# Autodesk Inventor assembly: 000 ASY GBK Gubkinskiy
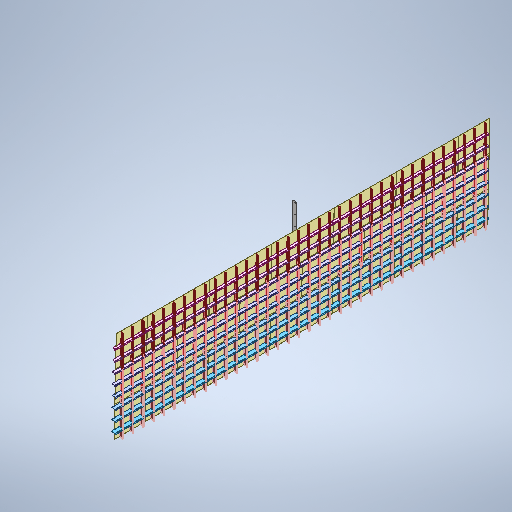
[picture p0: Inventor's stored thumbnail of the model, 512x512]
Saved by Autodesk Inventor 2026.2 (Build 302298000, 298)
## iProperties
Created: 2026-04-17
Part Number: 000 ASY GBK Gubkinskiy
Document SubType Name: Assembly
Designer: admin
Author: admin
## Documents named in this file (13)
- C:\Users\admin\Documents\Inventor\GBK-Gubkinskiy\000 ASY GBK Gubkinskiy.iam
- C:\Users\admin\Documents\Inventor\GBK-Gubkinskiy\GBK bottom.ipt
- C:\Users\admin\Documents\Inventor\GBK-Gubkinskiy\01 ASY GBK wall shield 1.1.1.iam
- C:\Users\admin\Documents\Inventor\GBK-Gubkinskiy\GBK dummy wall 1.ipt
- C:\Users\admin\Documents\Inventor\GBK-Gubkinskiy\GBK dummy wall 4.ipt
- C:\Users\admin\Documents\Inventor\GBK-Gubkinskiy\GBK overall model.ipt
- C:\Users\admin\Documents\Inventor\GBK-Gubkinskiy\02.1 GBK main rib.ipt
- C:\Users\admin\Documents\Inventor\GBK-Gubkinskiy\03.1 GBK main3  rib.ipt
- C:\Users\admin\Documents\Inventor\GBK-Gubkinskiy\02 ASY GBK wall shield 1.1.2.iam
- C:\Users\admin\Documents\Inventor\GBK-Gubkinskiy\04 ASY GBK wall shield 1.2.4.iam
- C:\Users\admin\Documents\Inventor\GBK-Gubkinskiy\07 ASY GBK wall shield 1.3.1.iam
- C:\Users\admin\Documents\Inventor\GBK-Gubkinskiy\08 ASY GBK wall shield 1.3.8.iam
- C:\Users\admin\Documents\Inventor\GBK-Gubkinskiy\0411 GBK Center main rib.ipt
## Components (28 placed, 13 different names)
1. GBK bottom.ipt:1 — Mate:10, Mate:11, Mate:12, Mate:13, Mate:14, Rigid:1
2. 01 ASY GBK wall shield 1.1.1.iam:1 [sub-assembly] — Rigid:4, Rigid:5
3. GBK dummy wall 1.ipt:1 — Mate:10
4. GBK dummy wall 1.ipt:2 — Mate:11, Mate:12
5. GBK dummy wall 4.ipt:1 — Mate:13, Mate:14
6. GBK overall model:1 — Rigid:1
7. 02.1 GBK main rib:1 — Rigid:3
8. 03.1 GBK main3  rib:1 — Rigid:3
9. 02 ASY GBK wall shield 1.1.2:1 [sub-assembly] — Rigid:4, Rigid:17
10. 04 ASY GBK wall shield 1.2.4:1 [sub-assembly] — Rigid:5, Rigid:6, Rigid:12
11. 07 ASY GBK wall shield 1.3.1:1 [sub-assembly] — Rigid:6, Rigid:7
12. 08 ASY GBK wall shield 1.3.8:1 [sub-assembly] — Rigid:7, Rigid:8
13. 08 ASY GBK wall shield 1.3.8:2 [sub-assembly] — Rigid:8, Rigid:9
14. 08 ASY GBK wall shield 1.3.8:3 [sub-assembly] — Rigid:9, Rigid:10
15. 08 ASY GBK wall shield 1.3.8:4 [sub-assembly] — Rigid:10, Rigid:11
16. 08 ASY GBK wall shield 1.3.8:5 [sub-assembly] — Rigid:11, Rigid:22
17. 04 ASY GBK wall shield 1.2.4:2 [sub-assembly] — Rigid:12, Rigid:13
18. 04 ASY GBK wall shield 1.2.4:3 [sub-assembly] — Rigid:13, Rigid:14
19. 04 ASY GBK wall shield 1.2.4:4 [sub-assembly] — Rigid:14, Rigid:15
20. 04 ASY GBK wall shield 1.2.4:5 [sub-assembly] — Rigid:15, Rigid:16
21. 04 ASY GBK wall shield 1.2.4:6 [sub-assembly] — Rigid:16
22. 02 ASY GBK wall shield 1.1.2:2 [sub-assembly] — Rigid:17, Rigid:18
23. 02 ASY GBK wall shield 1.1.2:3 [sub-assembly] — Rigid:18, Rigid:19
24. 02 ASY GBK wall shield 1.1.2:4 [sub-assembly] — Rigid:19, Rigid:20
25. 02 ASY GBK wall shield 1.1.2:5 [sub-assembly] — Rigid:20, Rigid:21
26. 01 ASY GBK wall shield 1.1.1:2 [sub-assembly] — Rigid:21
27. 07 ASY GBK wall shield 1.3.1:2 [sub-assembly] — Rigid:22
28. 0411 GBK Center main rib:1
## Relationships (30: WeldJoint 21, Mate 6, Flush 2, RevoluteJoint 1)
- [Flush]: GBK bottom.ipt:1 ↔ 01 ASY GBK wall shield 1.1.1.iam:1
- [Mate]: GBK bottom.ipt:1 ↔ 01 ASY GBK wall shield 1.1.1.iam:1
- Mate:10: GBK bottom.ipt:1 ↔ GBK dummy wall 1.ipt:1
- Mate:11: GBK bottom.ipt:1 ↔ GBK dummy wall 1.ipt:2
- Mate:12: GBK bottom.ipt:1 ↔ GBK dummy wall 1.ipt:2
- Mate:13: GBK bottom.ipt:1 ↔ GBK dummy wall 4.ipt:1
- Mate:14: GBK bottom.ipt:1 ↔ GBK dummy wall 4.ipt:1
- Rigid:1 [WeldJoint]: GBK bottom.ipt:1 ↔ GBK overall model:1
- [RevoluteJoint]: 01 ASY GBK wall shield 1.1.1.iam:1 ↔ 02.1 GBK main rib:1
- Rigid:3 [WeldJoint]: 02.1 GBK main rib:1 ↔ 03.1 GBK main3  rib:1
- [Flush]: 01 ASY GBK wall shield 1.1.1.iam:1 ↔ 02.1 GBK main rib:1
- Rigid:4 [WeldJoint] (1 mm): 01 ASY GBK wall shield 1.1.1.iam:1 ↔ 02 ASY GBK wall shield 1.1.2:1
- Rigid:5 [WeldJoint]: 01 ASY GBK wall shield 1.1.1.iam:1 ↔ 04 ASY GBK wall shield 1.2.4:1
- Rigid:6 [WeldJoint]: 04 ASY GBK wall shield 1.2.4:1 ↔ 07 ASY GBK wall shield 1.3.1:1
- Rigid:7 [WeldJoint] (1 mm): 07 ASY GBK wall shield 1.3.1:1 ↔ 08 ASY GBK wall shield 1.3.8:1
- Rigid:8 [WeldJoint] (1 mm): 08 ASY GBK wall shield 1.3.8:1 ↔ 08 ASY GBK wall shield 1.3.8:2
- Rigid:9 [WeldJoint] (1 mm): 08 ASY GBK wall shield 1.3.8:2 ↔ 08 ASY GBK wall shield 1.3.8:3
- Rigid:10 [WeldJoint] (1 mm): 08 ASY GBK wall shield 1.3.8:3 ↔ 08 ASY GBK wall shield 1.3.8:4
- Rigid:11 [WeldJoint] (1 mm): 08 ASY GBK wall shield 1.3.8:4 ↔ 08 ASY GBK wall shield 1.3.8:5
- Rigid:12 [WeldJoint] (1 mm): 04 ASY GBK wall shield 1.2.4:1 ↔ 04 ASY GBK wall shield 1.2.4:2
- Rigid:13 [WeldJoint] (1 mm): 04 ASY GBK wall shield 1.2.4:2 ↔ 04 ASY GBK wall shield 1.2.4:3
- Rigid:14 [WeldJoint] (1 mm): 04 ASY GBK wall shield 1.2.4:3 ↔ 04 ASY GBK wall shield 1.2.4:4
- Rigid:15 [WeldJoint] (1 mm): 04 ASY GBK wall shield 1.2.4:4 ↔ 04 ASY GBK wall shield 1.2.4:5
- Rigid:16 [WeldJoint] (1 mm): 04 ASY GBK wall shield 1.2.4:5 ↔ 04 ASY GBK wall shield 1.2.4:6
- Rigid:17 [WeldJoint] (1 mm): 02 ASY GBK wall shield 1.1.2:1 ↔ 02 ASY GBK wall shield 1.1.2:2
- Rigid:18 [WeldJoint] (1 mm): 02 ASY GBK wall shield 1.1.2:2 ↔ 02 ASY GBK wall shield 1.1.2:3
- Rigid:19 [WeldJoint] (1 mm): 02 ASY GBK wall shield 1.1.2:3 ↔ 02 ASY GBK wall shield 1.1.2:4
- Rigid:20 [WeldJoint] (1 mm): 02 ASY GBK wall shield 1.1.2:4 ↔ 02 ASY GBK wall shield 1.1.2:5
- Rigid:21 [WeldJoint] (1 mm): 02 ASY GBK wall shield 1.1.2:5 ↔ 01 ASY GBK wall shield 1.1.1:2
- Rigid:22 [WeldJoint] (1 mm): 08 ASY GBK wall shield 1.3.8:5 ↔ 07 ASY GBK wall shield 1.3.1:2
## Named parameters: Зазор_по_горизонту = 1 mm
